# Autodesk Inventor assembly: 2 in compliant wheel + clamping hub
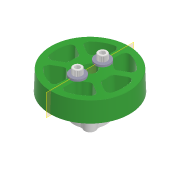
[picture p0: Inventor's stored thumbnail of the model, 180x180]
Saved by Autodesk Inventor 2020 (Build 240168000, 168)
## iProperties
Created: 2020-09-28
Part Number: 2 in compliant wheel + clamping hub
Document SubType Name: Assembly
Designer: ball
Author: ball
## Documents named in this file (7)
- C:\FTC\FTC8863CAD\2020 Robot\2 in compliant wheel + clamping hub.iam
- C:\FTC\FTC8863CAD\Actobotics\545 parts\545619 assembly.ipt
- C:\FTC\FTC8863CAD\Actobotics\545 parts\545456.ipt
- C:\FTC\FTC8863CAD\Andymark\am-3572 2IN 8mm Compliant Wheel REV2.ipt
- C:\FTC\FTC8863CAD\StepLibraries\Screws\6-32x.375 SOCKET HEAD CAP SCREW.ipt
- C:\FTC\FTC8863CAD\StepLibraries\Washers\6 washer.ipt
- C:\FTC\FTC8863CAD\StepLibraries\Screws\6-32x.750 SOCKET HEAD CAP SCREW.ipt
## Components (9 placed, 6 different names)
1. 545619 assembly:1 — Mate:1, Mate:2, Mate:3
2. 545456:1 — Mate:1, Mate:2, Mate:3, Mate:4, Mate:5, Mate:6, Mate:7, Mate:8, Mate:9, Mate:10
3. am-3572 2IN 8mm Compliant Wheel REV2:1 — Mate:8, Mate:9, Mate:10, Mate:11, Mate:12, Mate:13, Mate:14
4. 6-32x.375 SOCKET HEAD CAP SCREW:1 — Mate:4, Mate:5
5. 6-32x.375 SOCKET HEAD CAP SCREW:2 — Mate:6, Mate:7
6. 6 washer:1 — Mate:12, Mate:13, Mate:15, Mate:16
7. 6 washer:2 — Mate:11, Mate:14, Mate:17, Mate:18
8. 6-32x.750 SOCKET HEAD CAP SCREW:1 — Mate:17, Mate:18
9. 6-32x.750 SOCKET HEAD CAP SCREW:2 — Mate:15, Mate:16
## Relationships (18: Mate 18)
- Mate:1: 545619 assembly:1 ↔ 545456:1
- Mate:2: 545619 assembly:1 ↔ 545456:1
- Mate:3: 545619 assembly:1 ↔ 545456:1
- Mate:4: 545456:1 ↔ 6-32x.375 SOCKET HEAD CAP SCREW:1
- Mate:5: 545456:1 ↔ 6-32x.375 SOCKET HEAD CAP SCREW:1
- Mate:6: 545456:1 ↔ 6-32x.375 SOCKET HEAD CAP SCREW:2
- Mate:7: 545456:1 ↔ 6-32x.375 SOCKET HEAD CAP SCREW:2
- Mate:8: 545456:1 ↔ am-3572 2IN 8mm Compliant Wheel REV2:1
- Mate:9: 545456:1 ↔ am-3572 2IN 8mm Compliant Wheel REV2:1
- Mate:10: 545456:1 ↔ am-3572 2IN 8mm Compliant Wheel REV2:1
- Mate:11: am-3572 2IN 8mm Compliant Wheel REV2:1 ↔ 6 washer:2
- Mate:12: am-3572 2IN 8mm Compliant Wheel REV2:1 ↔ 6 washer:1
- Mate:13: am-3572 2IN 8mm Compliant Wheel REV2:1 ↔ 6 washer:1
- Mate:14: am-3572 2IN 8mm Compliant Wheel REV2:1 ↔ 6 washer:2
- Mate:15: 6 washer:1 ↔ 6-32x.750 SOCKET HEAD CAP SCREW:2
- Mate:16: 6 washer:1 ↔ 6-32x.750 SOCKET HEAD CAP SCREW:2
- Mate:17: 6 washer:2 ↔ 6-32x.750 SOCKET HEAD CAP SCREW:1
- Mate:18: 6 washer:2 ↔ 6-32x.750 SOCKET HEAD CAP SCREW:1
